# Autodesk Inventor assembly: RightMecanum-SubAssem01
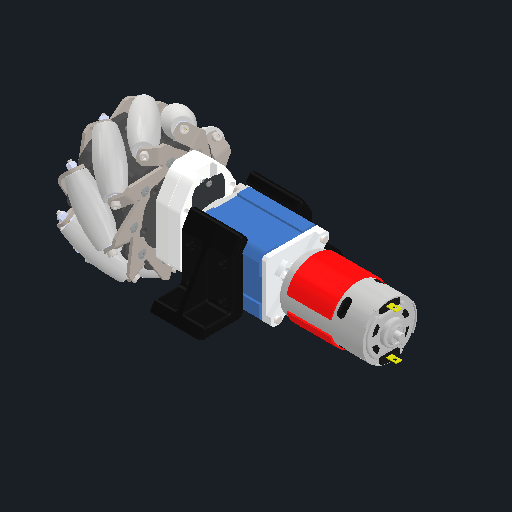
[picture p0: Inventor's stored thumbnail of the model, 512x512]
Saved by Autodesk Inventor 2024 (Build 280153000, 153)
## iProperties
Created: 2022-07-11
Part Number: RightMecanum-SubAssem01
Document SubType Name: Assembly
Designer: Dave
Author: Dave
## Documents named in this file (7)
- C:\Autodesk\ChalkBot Github\ChalkbotMechanical\Chalkbot1.0\Chassis\V1\RightMecanum-SubAssem01.iam
- C:\Autodesk\ChalkBot Github\ChalkbotMechanical\Chalkbot1.0\Chassis\V1\Mechanum STEP files\am-3775a AndyMark RedLine Motor (1).ipt
- C:\Autodesk\ChalkBot Github\ChalkbotMechanical\Chalkbot1.0\Chassis\V1\Motor and Gearbox STEP files\Hex Bore Mag Encoder Housing (217-6785).iam
- C:\Autodesk\ChalkBot Github\ChalkbotMechanical\Chalkbot1.0\Chassis\V1\Motor and Gearbox STEP files\am-3791 - 3000 x 500 Hex Shaft.ipt
- C:\Autodesk\ChalkBot Github\ChalkbotMechanical\Chalkbot1.0\Chassis\V1\Motor and Gearbox STEP files\2 Stage HD - 57 Sport.ipt
- C:\Autodesk\ChalkBot Github\ChalkbotMechanical\Chalkbot1.0\Chassis\V1\Mechanum STEP files\am-3918L 4HD 500H Mecanum Right.iam
- C:\Autodesk\ChalkBot Github\ChalkbotMechanical\Chalkbot1.0\Chassis\V1\Motor Mounts.ipt
## Components (7 placed, 6 different names)
1. 2 Stage HD - 57 Sport:1 — Insert:4, Insert:5, Angle:1, Mate:10, Insert:6, Insert:7, Insert:8, Insert:9
2. am-3775a AndyMark RedLine Motor (1):1 — Mate:9, Insert:5
3. Hex Bore Mag Encoder Housing (217-6785):1 [sub-assembly] — Mate:9, Mate:10
4. am-3791 - 3000 x 500 Hex Shaft:1 — Insert:4, Mate:11, Flush:1, Mate:12
5. am-3918L 4HD 500H Mecanum Right:1 [sub-assembly] — Mate:11, Flush:1, Mate:12
6. Motor Mounts:1 — Insert:6, Insert:7
7. Motor Mounts:2 — Insert:8, Insert:9
## Relationships (15: Insert 9, Mate 4, Angle 1, Flush 1)
- [Insert]: 2 Stage HD - 57 Sport:1 ↔ am-3775a AndyMark RedLine Motor (1):1
- [Insert]: 2 Stage HD - 57 Sport:1 ↔ am-3775a AndyMark RedLine Motor (1):1
- [Insert]: 2 Stage HD - 57 Sport:1 ↔ am-3791 - 3000 x 500 Hex Shaft:1
- Insert:4: 2 Stage HD - 57 Sport:1 ↔ am-3791 - 3000 x 500 Hex Shaft:1
- Mate:9: am-3775a AndyMark RedLine Motor (1):1 ↔ Hex Bore Mag Encoder Housing (217-6785):1
- Insert:5: 2 Stage HD - 57 Sport:1 ↔ am-3775a AndyMark RedLine Motor (1):1
- Angle:1 (0 deg): 2 Stage HD - 57 Sport:1
- Mate:10: 2 Stage HD - 57 Sport:1 ↔ Hex Bore Mag Encoder Housing (217-6785):1
- Mate:11: am-3791 - 3000 x 500 Hex Shaft:1 ↔ am-3918L 4HD 500H Mecanum Right:1
- Flush:1: am-3791 - 3000 x 500 Hex Shaft:1 ↔ am-3918L 4HD 500H Mecanum Right:1
- Mate:12: am-3791 - 3000 x 500 Hex Shaft:1 ↔ am-3918L 4HD 500H Mecanum Right:1
- Insert:6: 2 Stage HD - 57 Sport:1 ↔ Motor Mounts:1
- Insert:7: 2 Stage HD - 57 Sport:1 ↔ Motor Mounts:1
- Insert:8: 2 Stage HD - 57 Sport:1 ↔ Motor Mounts:2
- Insert:9: 2 Stage HD - 57 Sport:1 ↔ Motor Mounts:2
